# Autodesk Inventor assembly: Micro_Mate-N-Lok_TE-Connectivity_3mm_1x4_Male
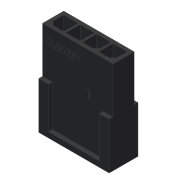
[picture p0: Inventor's stored thumbnail of the model, 180x180]
Saved by Autodesk Inventor 2015 (Build 190159000, 159)
## iProperties
Created: 2015-01-30
Part Number: Micro_Mate-N-Lok_TE-Connectivity_3mm_1x4_Male
Document SubType Name: Assembly
## Documents named in this file (3)
- C:\Dropbox\Inventor\Projects\001_EK-Teile\Micro_Mate-N-Lok_TE-Connectivity_3mm_1x4_Male.iam
- C:\Dropbox\Inventor\Projects\001_EK-Teile\Micro_Mate-N-Lok_TE-Connectivity_3mm_1x4_Male_1445049-4.ipt
- C:\Dropbox\Inventor\Projects\001_EK-Teile\Micro_Mate-N-Lok_TE-Connectivity_3mm_Crimp-Pin_1-794612-0.ipt
## Components (5 placed, 2 different names)
1. Micro_Mate-N-Lok_TE-Connectivity_3mm_1x4_Male_1445049-4:1 — Flush:2, Mate:2, Flush:1
2. Micro_Mate-N-Lok_TE-Connectivity_3mm_Crimp-Pin_1-794612-0:1 — Flush:2, Mate:2, Flush:1
3. Micro_Mate-N-Lok_TE-Connectivity_3mm_Crimp-Pin_1-794612-0:2
4. Micro_Mate-N-Lok_TE-Connectivity_3mm_Crimp-Pin_1-794612-0:3
5. Micro_Mate-N-Lok_TE-Connectivity_3mm_Crimp-Pin_1-794612-0:4
## Component patterns: (4 elements, first: Micro_Mate-N-Lok_TE-Connectivity_3mm_Crimp-Pin_1-794612-0:1)
## Relationships (3: Flush 2, Mate 1)
- Flush:2 (1.05 mm): Micro_Mate-N-Lok_TE-Connectivity_3mm_1x4_Male_1445049-4:1 ↔ Micro_Mate-N-Lok_TE-Connectivity_3mm_Crimp-Pin_1-794612-0:1
- Mate:2 (1.13 mm): Micro_Mate-N-Lok_TE-Connectivity_3mm_1x4_Male_1445049-4:1 ↔ Micro_Mate-N-Lok_TE-Connectivity_3mm_Crimp-Pin_1-794612-0:1
- Flush:1 (-0.1 mm): Micro_Mate-N-Lok_TE-Connectivity_3mm_1x4_Male_1445049-4:1 ↔ Micro_Mate-N-Lok_TE-Connectivity_3mm_Crimp-Pin_1-794612-0:1
